# Autodesk Inventor assembly: 스위치 조립품
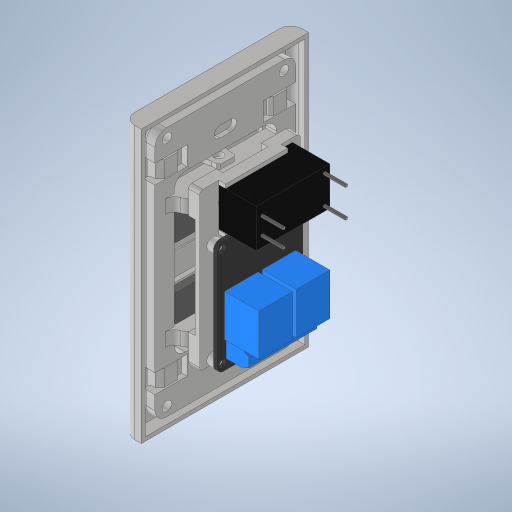
[picture p0: Inventor's stored thumbnail of the model, 512x512]
Saved by Autodesk Inventor 2023 (Build 270158000, 158)
## iProperties
Created: 2022-06-24
Part Number: 스위치 조립품
Document SubType Name: Assembly
Designer: user
Author: user
## Documents named in this file (10)
- C:\Users\user\Desktop\PAI\IOT부품\조명 스위치 2단\스위치 조립품.iam
- C:\Users\user\Desktop\PAI\IOT부품\조명 스위치 2단\조명 케이스.ipt
- C:\Users\user\Desktop\PAI\IOT부품\조명 스위치 2단\스위치 커버.ipt
- C:\Users\user\Desktop\PAI\IOT부품\esp32f.ipt
- C:\Users\user\Desktop\PAI\IOT부품\텍트 스위치.ipt
- C:\Users\user\Desktop\PAI\IOT부품\GMS0205.ipt
- C:\Users\user\Desktop\PAI\IOT부품\조명 스위치 2단\와이파이 모듈 커버.ipt
- C:\Users\user\Desktop\PAI\IOT부품\조명 스위치 2단\버튼 스위치 상단.ipt
- C:\Users\user\Desktop\PAI\IOT부품\조명 스위치 2단\버튼 스위치 하단.ipt
- C:\Users\user\Desktop\PAI\IOT부품\더블 릴레이 모듈.ipt
## Components (12 placed, 9 different names)
1. 조명 케이스:1 — 삽입:1, 삽입:2, 삽입:5, 삽입:6, 삽입:7, 삽입:8, 삽입:9, 삽입:10
2. 스위치 커버:1
3. esp32f:1 — 삽입:1, 삽입:2, 삽입:3, 삽입:4
4. 텍트 스위치:1 — 삽입:7
5. 텍트 스위치:2 — 삽입:8
6. GMS0205:1 — 메이트:4, 메이트:5
7. 와이파이 모듈 커버:1 — 삽입:3, 삽입:4, 메이트:4, 메이트:5, 삽입:11, 삽입:12
8. 텍트 스위치:3 — 삽입:5
9. 텍트 스위치:4 — 삽입:6
10. 버튼 스위치 상단:1 — 삽입:9
11. 버튼 스위치 하단:1 — 삽입:10
12. 더블 릴레이 모듈:1 — 삽입:11, 삽입:12
## Relationships (14: Insert 12, Mate 2)
- 삽입:1 [Insert]: 조명 케이스:1 ↔ esp32f:1
- 삽입:2 [Insert]: 조명 케이스:1 ↔ esp32f:1
- 삽입:3 [Insert]: esp32f:1 ↔ 와이파이 모듈 커버:1
- 삽입:4 [Insert]: esp32f:1 ↔ 와이파이 모듈 커버:1
- 메이트:4 [Mate]: GMS0205:1 ↔ 와이파이 모듈 커버:1
- 삽입:5 [Insert]: 조명 케이스:1 ↔ 텍트 스위치:3
- 삽입:6 [Insert]: 조명 케이스:1 ↔ 텍트 스위치:4
- 삽입:7 [Insert]: 조명 케이스:1 ↔ 텍트 스위치:1
- 삽입:8 [Insert]: 조명 케이스:1 ↔ 텍트 스위치:2
- 삽입:9 [Insert]: 조명 케이스:1 ↔ 버튼 스위치 상단:1
- 삽입:10 [Insert]: 조명 케이스:1 ↔ 버튼 스위치 하단:1
- 메이트:5 [Mate]: GMS0205:1 ↔ 와이파이 모듈 커버:1
- 삽입:11 [Insert]: 와이파이 모듈 커버:1 ↔ 더블 릴레이 모듈:1
- 삽입:12 [Insert]: 와이파이 모듈 커버:1 ↔ 더블 릴레이 모듈:1
